# Autodesk Inventor assembly: Type 1A 總組合 組合1
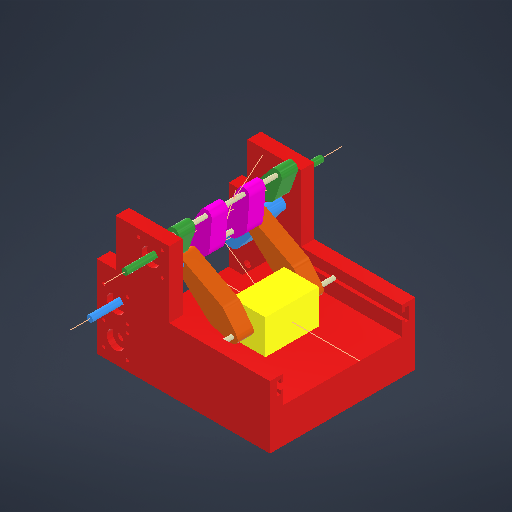
[picture p0: Inventor's stored thumbnail of the model, 512x512]
Saved by Autodesk Inventor 2025.3 (Build 293356030, 356C)
## iProperties
RuleStatus: InUse
Created: 2024-09-21
Part Number: Type 1A 總組合 組合1
Document SubType Name: Assembly
Designer: veter
Mass: 2.9492e+06 g
Surface Area: 86175 cm^2
Volume: 375694 cm^3
Density: 7.84999 g/cm^3
Author: veter
## Documents named in this file (8)
- C:\Users\Ou918\Downloads\AI-optimization\reference\model\Type 1A 總組合 組合1_modified.iam
- C:\Users\Ou918\Downloads\AI-optimization\reference\model\Type 1A R1前充座.ipt
- C:\Users\Ou918\Downloads\AI-optimization\reference\model\Type 1A R2延伸曲柄.ipt
- C:\Users\Ou918\Downloads\AI-optimization\reference\model\Type 1A R3延伸連接桿.ipt
- C:\Users\Ou918\Downloads\AI-optimization\reference\model\Type 1A R4主滑台曲柄.ipt
- C:\Users\Ou918\Downloads\AI-optimization\reference\model\Type 1A R5主滑台連接桿.ipt
- C:\Users\Ou918\Downloads\AI-optimization\reference\model\Type 1A 連接軸 1.ipt
- C:\Users\Ou918\Downloads\AI-optimization\reference\model\Type 1A R6主滑台_modified.ipt
## Components (9 placed, 7 different names)
1. Type 1A R1前充座:1 — J12, J14, 滑塊:1
2. Type 1A R2延伸曲柄:1 — J12, 剛性:1, J23, 角度:1
3. Type 1A R3延伸連接桿:1 — J34, J23, J35
4. Type 1A R4主滑台曲柄:1 — J14, 剛性:2, J34, J45
5. Type 1A R5主滑台連接桿:1 — J35, J45, 圓柱:4, 貼合:1
6. Type 1A R6主滑台_modified:1 — 滑塊:1, 圓柱:5
7. Type 1A 連接軸 1:7 — 剛性:1
8. Type 1A 連接軸 1:8 — 剛性:2
9. Type 1A 連接軸 1:9 — 圓柱:4, 圓柱:5, 貼合:1
## Relationships (13: RevoluteJoint 4, CylindricalJoint 4, WeldJoint 2, Angle 1, TranslationJoint 1, Mate 1)
- J12 [RevoluteJoint]: Type 1A R1前充座:1 ↔ Type 1A R2延伸曲柄:1
- J14 [RevoluteJoint]: Type 1A R1前充座:1 ↔ Type 1A R4主滑台曲柄:1
- J23 [CylindricalJoint]: Type 1A R2延伸曲柄:1 ↔ Type 1A R3延伸連接桿:1
- J34 [RevoluteJoint] (-103 mm): Type 1A R3延伸連接桿:1 ↔ Type 1A R4主滑台曲柄:1
- J35 [CylindricalJoint]: Type 1A R3延伸連接桿:1 ↔ Type 1A R5主滑台連接桿:1
- J45 [RevoluteJoint]: Type 1A R4主滑台曲柄:1 ↔ Type 1A R5主滑台連接桿:1
- 剛性:1 [WeldJoint]: Type 1A R2延伸曲柄:1 ↔ Type 1A 連接軸 1:7
- 剛性:2 [WeldJoint]: Type 1A R4主滑台曲柄:1 ↔ Type 1A 連接軸 1:8
- 角度:1 [Angle] (89 deg): Type 1A R2延伸曲柄:1
- 圓柱:4 [CylindricalJoint]: Type 1A R5主滑台連接桿:1 ↔ Type 1A 連接軸 1:9
- 滑塊:1 [TranslationJoint]: Type 1A R1前充座:1 ↔ Type 1A R6主滑台_modified:1
- 圓柱:5 [CylindricalJoint]: Type 1A R6主滑台_modified:1 ↔ Type 1A 連接軸 1:9
- 貼合:1 [Mate]: Type 1A R5主滑台連接桿:1 ↔ Type 1A 連接軸 1:9
## Named parameters: con_th = 45 deg
